# Autodesk Inventor assembly: BatteryDrawer
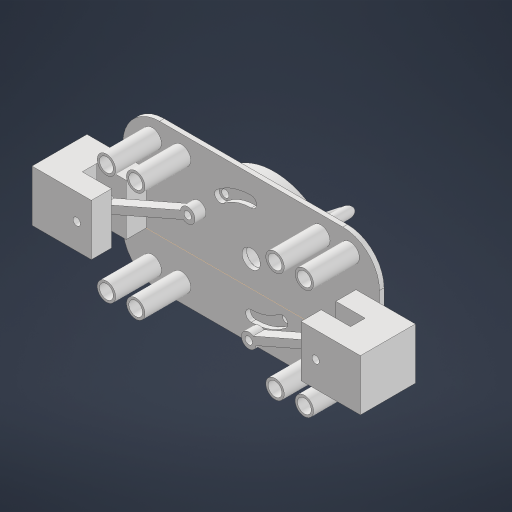
[picture p0: Inventor's stored thumbnail of the model, 512x512]
Saved by Autodesk Inventor 2024 (Build 280153000, 153)
## iProperties
Created: 2024-01-21
Part Number: BatteryDrawer
Document SubType Name: Assembly
Designer: Nebil Oumer
Author: Nebil Oumer
## Documents named in this file (7)
- C:\Users\calvi\OneDrive\Robocup Rescue\Chassis\Battery Drawer\BatteryDrawer.iam
- C:\Users\calvi\OneDrive\Robocup Rescue\Chassis\Battery Drawer\Slider.ipt
- C:\Users\calvi\OneDrive\Robocup Rescue\Chassis\Battery Drawer\Crank.ipt
- C:\Users\calvi\OneDrive\Robocup Rescue\Chassis\Battery Drawer\Plate.ipt
- C:\Users\calvi\OneDrive\Robocup Rescue\Chassis\Battery Drawer\Beam.ipt
- C:\Users\calvi\OneDrive\Robocup Rescue\Chassis\Battery Drawer\Handle.ipt
- C:\Users\calvi\OneDrive\Robocup Rescue\Chassis\Battery Drawer\RCR_Battery_Drawer_Bearings\RCR_Battery_Drawer_Bearings.ipt
## Components (15 placed, 6 different names)
1. Slider:2 — Mate:3, Mate:4, Mate:10, Flush:1
2. Crank:1 — Mate:8, Mate:9, Mate:14, Mate:18, Mate:19, Mate:20, Rigid:1
3. Plate:1 — Mate:4, Mate:8, Flush:1, Mate:15, Flush:2, Mate:18, Rotational:3, Rotational:4, Rotational:5, Rotational:6, Rotational:7, Rotational:8, Rotational:9, Rotational:10
4. Beam:1 — Mate:3, Mate:9, Mate:10
5. Beam:2 — Mate:14, Mate:16, Mate:17
6. Handle:1 — Mate:19, Mate:20, Rigid:1
7. Slider:3 — Mate:15, Mate:16, Mate:17, Flush:2
8. RCR_Battery_Drawer_Bearings:1 — Rotational:7
9. RCR_Battery_Drawer_Bearings:2 — Rotational:8
10. RCR_Battery_Drawer_Bearings:3 — Rotational:9
11. RCR_Battery_Drawer_Bearings:4 — Rotational:10
12. RCR_Battery_Drawer_Bearings:5 — Rotational:6
13. RCR_Battery_Drawer_Bearings:6 — Rotational:3
14. RCR_Battery_Drawer_Bearings:7 — Rotational:5
15. RCR_Battery_Drawer_Bearings:8 — Rotational:4
## Relationships (23: Mate 12, RevoluteJoint 8, Flush 2, WeldJoint 1)
- Mate:3: Slider:2 ↔ Beam:1
- Mate:4: Slider:2 ↔ Plate:1
- Mate:8: Crank:1 ↔ Plate:1
- Mate:9: Crank:1 ↔ Beam:1
- Mate:10 (1.27 mm): Slider:2 ↔ Beam:1
- Flush:1: Slider:2 ↔ Plate:1
- Mate:14: Crank:1 ↔ Beam:2
- Mate:15: Plate:1 ↔ Slider:3
- Mate:16: Beam:2 ↔ Slider:3
- Mate:17 (1.27 mm): Beam:2 ↔ Slider:3
- Flush:2: Plate:1 ↔ Slider:3
- Mate:18: Crank:1 ↔ Plate:1
- Mate:19: Crank:1 ↔ Handle:1
- Mate:20: Crank:1 ↔ Handle:1
- Rigid:1 [WeldJoint]: Crank:1 ↔ Handle:1
- Rotational:3 [RevoluteJoint]: Plate:1 ↔ RCR_Battery_Drawer_Bearings:6
- Rotational:4 [RevoluteJoint]: Plate:1 ↔ RCR_Battery_Drawer_Bearings:8
- Rotational:5 [RevoluteJoint]: Plate:1 ↔ RCR_Battery_Drawer_Bearings:7
- Rotational:6 [RevoluteJoint]: Plate:1 ↔ RCR_Battery_Drawer_Bearings:5
- Rotational:7 [RevoluteJoint]: Plate:1 ↔ RCR_Battery_Drawer_Bearings:1
- Rotational:8 [RevoluteJoint]: Plate:1 ↔ RCR_Battery_Drawer_Bearings:2
- Rotational:9 [RevoluteJoint]: Plate:1 ↔ RCR_Battery_Drawer_Bearings:3
- Rotational:10 [RevoluteJoint]: Plate:1 ↔ RCR_Battery_Drawer_Bearings:4
